# Autodesk Inventor assembly: Assembly2
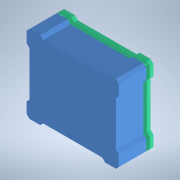
[picture p0: Inventor's stored thumbnail of the model, 180x180]
Saved by Autodesk Inventor 2020 (Build 240168000, 168)
## iProperties
Created: 2020-02-07
Part Number: Assembly2
Document SubType Name: Assembly
Designer: Alex
Author: Alex
## Documents named in this file (5)
- C:\Users\Alex\Documents\Inventor\Ventolino2\Assembly2.iam
- C:\Users\Alex\Documents\Inventor\Ventolino2\Case.ipt
- C:\Users\Alex\Documents\Inventor\Ventolino2\Lid.ipt
- C:\Users\Alex\Documents\Inventor\Ventolino2\ArduinoMEGA2560.ipt
- C:\Users\Alex\Documents\Inventor\Ventolino2\D-SUB.ipt
## Components (7 placed, 4 different names)
1. Case:1 — Flush:1, Rotational:1, Rotational:2, Rotational:3, Rotational:4, Rotational:5, Rotational:6, Mate:1
2. Lid:1 — Flush:2, Mate:1
3. -  -:1 — Rotational:1, Rotational:2
4. D-SUB:1 — Rotational:3
5. D-SUB:2 — Rotational:4
6. D-SUB:3 — Rotational:5
7. D-SUB:4 — Rotational:6
## Relationships (9: RevoluteJoint 6, Flush 2, Mate 1)
- Flush:1 (10 mm): Case:1
- Flush:2: Lid:1
- Rotational:1 [RevoluteJoint]: Case:1 ↔ -  -:1
- Rotational:2 [RevoluteJoint]: Case:1 ↔ -  -:1
- Rotational:3 [RevoluteJoint]: Case:1 ↔ D-SUB:1
- Rotational:4 [RevoluteJoint]: Case:1 ↔ D-SUB:2
- Rotational:5 [RevoluteJoint]: Case:1 ↔ D-SUB:3
- Rotational:6 [RevoluteJoint]: Case:1 ↔ D-SUB:4
- Mate:1: Case:1 ↔ Lid:1
